# Autodesk Inventor assembly: Emsable poyecto
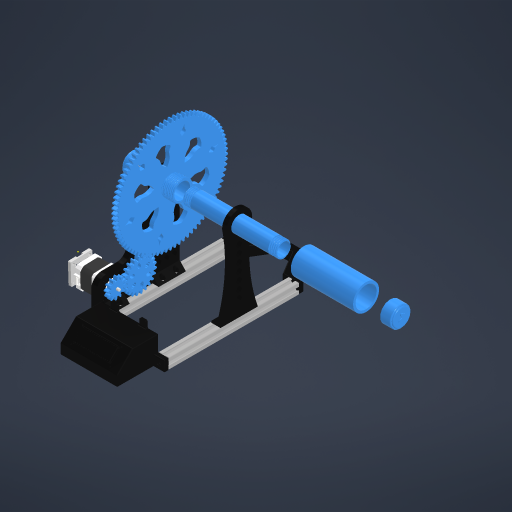
[picture p0: Inventor's stored thumbnail of the model, 512x512]
Saved by Autodesk Inventor 2023 (Build 270158000, 158)
## iProperties
Created: 2023-11-13
Part Number: Emsable poyecto
Document SubType Name: Assembly
Designer: danie
Author: danie
## Documents named in this file (15)
- C:\Users\danie\Downloads\ProyectoF (5)\ProyectoF\Emsable poyecto.iam
- C:\Users\danie\Downloads\ProyectoF (5)\ProyectoF\Extrusion 2020x10.ipt
- C:\Users\danie\Downloads\ProyectoF (5)\ProyectoF\Soporte.ipt
- C:\Users\danie\Downloads\ProyectoF (5)\ProyectoF\Holder.ipt
- C:\Users\danie\Downloads\ProyectoF (5)\ProyectoF\HolderB.ipt
- C:\Users\danie\Downloads\ProyectoF (5)\ProyectoF\NEMA17.ipt
- C:\Users\danie\Downloads\ProyectoF (5)\ProyectoF\Skate-Bearing.ipt
- C:\Users\danie\Downloads\ProyectoF (5)\ProyectoF\Cajita.iam
- C:\Users\danie\Downloads\ProyectoF (5)\ProyectoF\Spur Gear (12 teeth).ipt
- C:\Users\danie\Downloads\ProyectoF (5)\ProyectoF\Spur Gear (22 teeth).ipt
- C:\Users\danie\Downloads\ProyectoF (5)\ProyectoF\Spur Gear (80 teeth).ipt
- C:\Users\danie\Downloads\ProyectoF (5)\ProyectoF\Barra.ipt
- C:\Users\danie\Downloads\ProyectoF (5)\ProyectoF\Barrita.ipt
- C:\Users\danie\Downloads\ProyectoF (5)\ProyectoF\tapas.ipt
- C:\Users\danie\Downloads\ProyectoF (5)\ProyectoF\Soporte PCBs N17 V2.ipt
## Components (16 placed, 14 different names)
1. Extrusion 2020x10:1 — Mate:2, Flush:1, Mate:6, Mate:7, Mate:9, Mate:15, Mate:17, Angle:1, Flush:6, Mate:24
2. Extrusion 2020x10:2 — Mate:1, Flush:2, Mate:8, Mate:10, Mate:14, Flush:7
3. Soporte:2 — Mate:6, Mate:7, Mate:8
4. Holder:1 — Mate:9, Mate:11, Mate:12, Mate:13, Flush:3, Mate:18, Flush:6, Flush:10, Mate:30, Mate:31
5. HolderB:1 — Mate:10, Mate:19, Flush:7, Mate:29, Mate:30
6. NEMA17:1 — Mate:11, Mate:12, Mate:21, Flush:8, Mate:32, Mate:33
7. Skate-Bearing:1 — Mate:13, Mate:22, Flush:10
8. Cajita:1 [sub-assembly] — Mate:14, Mate:15, Mate:20
9. Spur Gear (12 teeth):1 — Mate:21, Flush:9, Rotation:1
10. Spur Gear (22 teeth):1 — Mate:22, Flush:11, Rotation:1, Rotation:2
11. Spur Gear (80 teeth):1 — Flush:12, Mate:31, Rotation:2
12. Barra:1 — Mate:26
13. Barrita:1 — Mate:26, Mate:27, Mate:28, Mate:29
14. tapas:1 — Mate:27
15. tapas:2 — Mate:28
16. Soporte PCBs N17 V2:1 — Mate:32, Mate:33
## Relationships (40: Mate 27, Flush 10, RelateRotation 2, Angle 1)
- Mate:1: Extrusion 2020x10:2
- Mate:2: Extrusion 2020x10:1
- Flush:1: Extrusion 2020x10:1
- Flush:2: Extrusion 2020x10:2
- Mate:6: Extrusion 2020x10:1 ↔ Soporte:2
- Mate:7: Extrusion 2020x10:1 ↔ Soporte:2
- Mate:8: Extrusion 2020x10:2 ↔ Soporte:2
- Mate:9: Extrusion 2020x10:1 ↔ Holder:1
- Mate:10: Extrusion 2020x10:2 ↔ HolderB:1
- Mate:11: Holder:1 ↔ NEMA17:1
- Mate:12: Holder:1 ↔ NEMA17:1
- Mate:13: Holder:1 ↔ Skate-Bearing:1
- Mate:14: Extrusion 2020x10:2 ↔ Cajita:1
- Mate:15: Extrusion 2020x10:1 ↔ Cajita:1
- Mate:17: Extrusion 2020x10:1
- Angle:1 (0 deg): Extrusion 2020x10:1
- Flush:3: Holder:1
- Mate:18: Holder:1
- Mate:19: HolderB:1
- Mate:20: Cajita:1
- Flush:6: Extrusion 2020x10:1 ↔ Holder:1
- Flush:7: Extrusion 2020x10:2 ↔ HolderB:1
- Mate:21: NEMA17:1 ↔ Spur Gear (12 teeth):1
- Mate:22: Skate-Bearing:1 ↔ Spur Gear (22 teeth):1
- Flush:8 (-5 mm): NEMA17:1
- Flush:9: Spur Gear (12 teeth):1
- Mate:24: Extrusion 2020x10:1
- Flush:10: Holder:1 ↔ Skate-Bearing:1
- Flush:11: Spur Gear (22 teeth):1
- Flush:12: Spur Gear (80 teeth):1
- Rotation:1 [RelateRotation] (0.5455 ul): Spur Gear (12 teeth):1 ↔ Spur Gear (22 teeth):1
- Mate:26: Barra:1 ↔ Barrita:1
- Mate:27: Barrita:1 ↔ tapas:1
- Mate:28: Barrita:1 ↔ tapas:2
- Mate:29: HolderB:1 ↔ Barrita:1
- Mate:30: Holder:1 ↔ HolderB:1
- Mate:31: Holder:1 ↔ Spur Gear (80 teeth):1
- Rotation:2 [RelateRotation] (0.275 ul): Spur Gear (22 teeth):1 ↔ Spur Gear (80 teeth):1
- Mate:32: NEMA17:1 ↔ Soporte PCBs N17 V2:1
- Mate:33: NEMA17:1 ↔ Soporte PCBs N17 V2:1
